# Autodesk Inventor assembly: lampara 54 leds
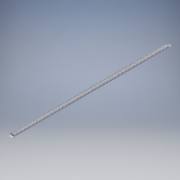
[picture p0: Inventor's stored thumbnail of the model, 180x180]
Saved by Autodesk Inventor 2017 (Build 210142000, 142)
## iProperties
Created: 2016-04-21
Part Number: lampara 54 leds
Document SubType Name: Assembly
Designer: umr
Sending System: SolidWorks 2016
Last Author: DETEC
Last Saved: 2016-06-10
Author: umr
## Documents named in this file (5)
- D:\SeniorProject\Models2\LED Tube\lampara 54 leds.iam
- D:\SeniorProject\Models2\LED Tube\disipador.ipt
- D:\SeniorProject\Models2\LED Tube\5cmLedStrip.iam
- D:\SeniorProject\Models2\LED Tube\tapa.ipt
- D:\SeniorProject\Models2\LED Tube\tapabase.ipt
## Components (22 placed, 4 different names)
1. disipador:1 — Mate:1, Flush:1, Flush:2
2. 5cmLedStrip:1 [sub-assembly]
3. 5cmLedStrip:2 [sub-assembly]
4. 5cmLedStrip:3 [sub-assembly]
5. 5cmLedStrip:4 [sub-assembly]
6. 5cmLedStrip:5 [sub-assembly]
7. 5cmLedStrip:6 [sub-assembly]
8. 5cmLedStrip:7 [sub-assembly]
9. 5cmLedStrip:8 [sub-assembly]
10. 5cmLedStrip:9 [sub-assembly]
11. 5cmLedStrip:10 [sub-assembly]
12. 5cmLedStrip:11 [sub-assembly]
13. 5cmLedStrip:12 [sub-assembly]
14. 5cmLedStrip:13 [sub-assembly]
15. 5cmLedStrip:14 [sub-assembly]
16. 5cmLedStrip:15 [sub-assembly]
17. 5cmLedStrip:16 [sub-assembly]
18. 5cmLedStrip:17 [sub-assembly]
19. 5cmLedStrip:18 [sub-assembly]
20. tapa:1
21. tapabase:1
22. tapabase:2 — Mate:1, Flush:1, Flush:2
## Relationships (3: Flush 2, Mate 1)
- Mate:1: disipador:1 ↔ tapabase:2
- Flush:1: disipador:1 ↔ tapabase:2
- Flush:2: disipador:1 ↔ tapabase:2
